# Autodesk Inventor assembly: door_assembly
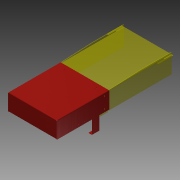
[picture p0: Inventor's stored thumbnail of the model, 180x180]
Saved by Autodesk Inventor 2014 SP2 (Build 180246200, 246)
## iProperties
Created: 2016-05-06
Part Number: door_assembly
Document SubType Name: Assembly
Designer: cruiser
Author: cruiser
## Documents named in this file (6)
- C:\Users\cruiser\Desktop\models\3d printers\laserresin4\door_assembly.iam
- C:\Users\cruiser\Desktop\models\3d printers\laserresin4\drawer.ipt
- C:\Users\cruiser\Desktop\models\3d printers\laserresin4\window.ipt
- C:\Users\cruiser\Desktop\models\3d printers\laserresin4\door.ipt
- C:\Users\cruiser\Desktop\models\3d printers\laserresin4\drawer_support.ipt
- C:\Users\cruiser\Desktop\models\3d printers\laserresin4\laserresin4.xlsx
## Components (5 placed, 4 different names)
1. drawer:1 — Mate:5, Mate:6, Mate:7, Mate:10, Mate:11, Mate:12, Mate:13, Mate:14, Mate:15, Mate:16, Flush:1, Mate:17
2. window:1 — Mate:7, Mate:14, Mate:15
3. window:2 — Mate:6, Mate:12, Mate:13
4. door:1 — Mate:5, Mate:10, Mate:11
5. drawer_support:1 — Mate:16, Flush:1, Mate:17
## Relationships (12: Mate 11, Flush 1)
- Mate:5: drawer:1 ↔ door:1
- Mate:6: drawer:1 ↔ window:2
- Mate:7: drawer:1 ↔ window:1
- Mate:10: drawer:1 ↔ door:1
- Mate:11: drawer:1 ↔ door:1
- Mate:12: drawer:1 ↔ window:2
- Mate:13: drawer:1 ↔ window:2
- Mate:14: drawer:1 ↔ window:1
- Mate:15: drawer:1 ↔ window:1
- Mate:16: drawer:1 ↔ drawer_support:1
- Flush:1 (48 mm): drawer:1 ↔ drawer_support:1
- Mate:17: drawer:1 ↔ drawer_support:1
## Named parameters: sm_thickness = 1.5875 mm, very_thick_acrylic = 9.45 mm, thick_acrylic = 5.88 mm, thin_acrylic = 3.15 mm, clear_acrylic = 3.15 mm, wood_thickness = 6.72 mm, m3_diameter = 3 mm, m4_diameter = 4 mm, m5_diameter = 5 mm, brass_insert_drill = 4 mm, m5_brass_insert_drill = 6.7 mm, m3_main_length = 14 mm, m3_main_nut_width = 5.7 mm, m3_main_nut_thickness = 2.5 mm, m3_main_extra = 1 mm, stepper_screw_space = 35 mm, stepper_shaft_diameter = 5 mm, stepper_body_diameter = 28 mm, laser_body_length = 40 mm, laser_body_diameter = 12 mm, carrier_x = 350 mm, carrier_y = 251 mm, carrier_z = 12 mm, visor_x = 257.3 mm, visor_y = 111.0625 mm, visor_overlap = 20 mm, protection_slot = 44.2 mm, protection_slot_offset = 55.25 mm, protection_slot_length = 80 mm, window_z = 333.9125 mm, window_y = 92.0625 mm, window_overlap = 48 mm, window_slot = 50 mm, window_frame_slot = 50 mm, door_x = 251 mm, door_z = 333.9125 mm, door_overlap = 48 mm, reservoir_x = 201 mm, reservoir_y = 201 mm, reservoir_z = 40 mm, reservoir_overlap = 20 mm, linear_bearing_spacing = 271 mm, linear_bearing_z = 400 mm, threaded_rod_z = 300 mm, motor_spacing = 337 mm, tray_border = 25 mm, tray_x = 251 mm, tray_y = 251 mm, bed_x = 150 mm, bed_y = 150 mm, bed_z = 25 mm, bed_z2 = 80 mm, stopper_diameter = 10 mm, crane_x = 330 mm, crane_y = 70 mm, crane_z = 60 mm, crane_z2 = 12 mm, end_stop_offset_x = 50 mm, end_stop_spacing = 19 mm, acrylic_into_frame = 5 mm, protection_slot_width = 10 mm, nema17_x = 43 mm, nema17_l = 60 mm, drawer_z = 278.175 mm, drawer_y = 88.65 mm, drawer_x = 257.3 mm, drawer_z_from_bottom = 25 mm, galvo_frame_z = 65 mm, galvo_frame_x = 66 mm, t_galvo_frame = 6.72 mm, galvo_frame_y_offset = 27.5 mm, laser_x = 30 mm, laser_z = 75 mm, laser_z_offset = 55 mm, laser_diameter = 12 mm, laser_y_offset = 19.4 mm, laser_y = 15 mm, subframe_z = 60 mm, subframe_x = 195 mm, subframe_y_offset = 27.5 mm, lcd_y = 25 mm, lcd_x = 72 mm, middle_frame_from_bottom = 150 mm, printer_z = 289 mm, bracket_z = 30 mm, frame_tilt = 1 deg, frame_foot_z = 12 mm, frame_border = 46.35 mm, printer_from_bottom = 200 mm, frame_z = 300 mm, frame_total_z = 661.5875 mm, frame_bottom_z = 275 mm, frame_top_z = 385 mm, frame_y = 80 mm, z_min_from_center = 115 mm, thumb_nut_diameter = 7 mm, thumb_nut_offset_y = 0 mm, m3_press_nut_drill = 4.5 mm, m3_head = 6 mm, m5_head = 10 mm, m5_press_nut_drill = 6.5 mm, drawer_support_overlap = 40 mm, drawer_support_from_top = 48 mm, laser_gap = 1 mm, frame_screw_from_center = 25 mm, galvo_frame_y = 20 mm, frame_magnet_offset = 20 mm, magnet_z = 50 mm, drawer_screw_z = 140 mm, drawer_screw_from_center = 54 mm, frame_face_y = 44 mm, magnet_screw_spacing = 30 mm, magnet_screw_from_edge = 10 mm, switch_spacing = 19 mm
